# Autodesk Inventor assembly: v.3
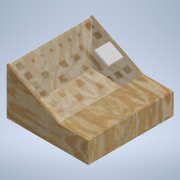
[picture p0: Inventor's stored thumbnail of the model, 180x180]
Saved by Autodesk Inventor 2021.1 (Build 251245000, 245)
## iProperties
Created: 2020-08-02
Part Number: v.3
Document SubType Name: Assembly
Designer: adick
Author: adick
## Documents named in this file (8)
- C:\Users\adick\Documents\Kerbal Kontroller\CAD\v.3.iam
- C:\Users\adick\Documents\Kerbal Kontroller\CAD\Parts\Sides.ipt
- C:\Users\adick\Documents\Kerbal Kontroller\CAD\Parts\Bottom.ipt
- C:\Users\adick\Documents\Kerbal Kontroller\CAD\Parts\Front.ipt
- C:\Users\adick\Documents\Kerbal Kontroller\CAD\Parts\Back.ipt
- C:\Users\adick\Documents\Kerbal Kontroller\CAD\Parts\Plexi.ipt
- C:\Users\adick\Documents\Kerbal Kontroller\CAD\Parts\Arm Rest.ipt
- C:\Users\adick\Documents\Kerbal Kontroller\CAD\Parts\Stage Keycap.ipt
## Components (8 placed, 7 different names)
1. Sides:1 — Mate:3, Mate:5, Mate:8, Mate:9, Mate:11
2. Bottom:1 — Mate:2, Mate:10
3. Front:1 — Mate:1, Mate:9, Mate:10
4. Back:1 — Mate:11
5. Sides:2 — Mate:1, Mate:2, Mate:4
6. Plexi:1 — Mate:3, Mate:4, Mate:5, Mate:6, Mate:7, Mate:12
7. Arm Rest:1 — Mate:8
8. Stage Keycap:1 — Mate:6, Mate:7, Mate:12
## Relationships (12: Mate 12)
- Mate:1: Front:1 ↔ Sides:2
- Mate:2: Bottom:1 ↔ Sides:2
- Mate:3: Sides:1 ↔ Plexi:1
- Mate:4: Sides:2 ↔ Plexi:1
- Mate:5: Sides:1 ↔ Plexi:1
- Mate:6: Plexi:1 ↔ Stage Keycap:1
- Mate:7: Plexi:1 ↔ Stage Keycap:1
- Mate:8: Sides:1 ↔ Arm Rest:1
- Mate:9: Sides:1 ↔ Front:1
- Mate:10: Bottom:1 ↔ Front:1
- Mate:11: Sides:1 ↔ Back:1
- Mate:12: Plexi:1 ↔ Stage Keycap:1
